# Autodesk Inventor assembly: Assembly_Cube_empty_IM_v3
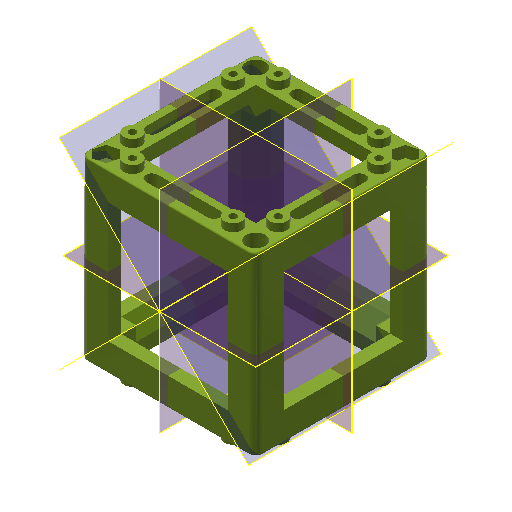
[picture p0: Inventor's stored thumbnail of the model, 512x512]
Saved by Autodesk Inventor 2023 (Build 270158000, 158)
## iProperties
Created: 2020-03-27
Part Number: Assembly_Cube_empty_IM_v3
Document SubType Name: Assembly
Designer: B
Mass: 22.3092 g
Surface Area: 188.369 cm^2
Volume: 22.3092 cm^3
Density: 1 g/cm^3
Author: B
## Documents named in this file (2)
- C:\Users\diederichbenedict\Downloads\UC2 setup design\UC2 setup design\Assembly_Cube_empty_IM_v3.iam
- C:\Users\diederichbenedict\Downloads\UC2 setup design\UC2 setup design\10_Cube_1x1_IM.ipt
## Components (2 placed, 1 different names)
1. 10_Cube_1x1_IM:1 — Angle:1, Mate:2, Symmetry:1, Symmetrie:2, Symmetrie:3, Symmetrie:4, Symmetrie:5, Symmetrie:6, Symmetrie:7
2. 10_Cube_1x1_IM:2 — Flush:1, Flush:2, Flush:3, Angle:1, Mate:2, Symmetry:1, Symmetrie:2, Symmetrie:3, Symmetrie:4, Symmetrie:5, Symmetrie:6, Symmetrie:7
## Relationships (16: Symmetry 7, Mate 5, Flush 3, Angle 1)
- Flush:1: 10_Cube_1x1_IM:2
- Flush:2: 10_Cube_1x1_IM:2
- Flush:3: 10_Cube_1x1_IM:2
- Angle:1 (0 deg): 10_Cube_1x1_IM:1 ↔ 10_Cube_1x1_IM:2
- Mate:2 (-50.1 mm): 10_Cube_1x1_IM:1 ↔ 10_Cube_1x1_IM:2
- Symmetry:1: 10_Cube_1x1_IM:1 ↔ 10_Cube_1x1_IM:2
- Symmetrie:2: 10_Cube_1x1_IM:1 ↔ 10_Cube_1x1_IM:2
- Symmetrie:3: 10_Cube_1x1_IM:1 ↔ 10_Cube_1x1_IM:2
- Symmetrie:4: 10_Cube_1x1_IM:1 ↔ 10_Cube_1x1_IM:2
- Symmetrie:5: 10_Cube_1x1_IM:1 ↔ 10_Cube_1x1_IM:2
- Symmetrie:6: 10_Cube_1x1_IM:1 ↔ 10_Cube_1x1_IM:2
- Symmetrie:7: 10_Cube_1x1_IM:1 ↔ 10_Cube_1x1_IM:2
- Mate:3
- Mate:4
- Mate:5
- Mate:6
